# Autodesk Inventor assembly: Center Assembly
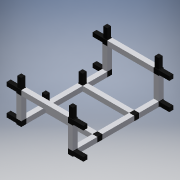
[picture p0: Inventor's stored thumbnail of the model, 180x180]
Saved by Autodesk Inventor 2017 (Build 210142000, 142)
## iProperties
Created: 2019-12-06
Part Number: Center Assembly
Document SubType Name: Assembly
Designer: S346553810
Author: S346553810
## Documents named in this file (9)
- \\ad.ocdsb.ca\studenthome\3\S338674153\FRC 2020\FullRobotRefactor\SubFrame\Center Assembly.iam
- \\ad.ocdsb.ca\studenthome\3\S338674153\FRC 2020\FullRobotRefactor\SubFrame\center cross-member.iam
- \\ad.ocdsb.ca\studenthome\3\S338674153\FRC 2020\FullRobotRefactor\SubFrame\1in sq tub - 4.ipt
- \\ad.ocdsb.ca\studenthome\3\S338674153\FRC 2020\FullRobotRefactor\SubFrame\Kipp K0619.ipt
- \\ad.ocdsb.ca\studenthome\3\S338674153\FRC 2020\FullRobotRefactor\SubFrame\1in sq tub - 6.ipt
- \\ad.ocdsb.ca\studenthome\3\S338674153\FRC 2020\FullRobotRefactor\SubFrame\1in sq tub - 4-5.ipt
- \\ad.ocdsb.ca\studenthome\3\S338674153\FRC 2020\FullRobotRefactor\SubFrame\1in sq tub - 6-5.ipt
- \\ad.ocdsb.ca\studenthome\3\S338674153\FRC 2020\FullRobotRefactor\KIPS\Kipp K0618.ipt
- \\ad.ocdsb.ca\studenthome\3\S338674153\FRC 2020\FullRobotRefactor\KIPS\Kipp K0620.ipt
## Components (14 placed, 8 different names)
1. center cross-member:1 [sub-assembly] — Flush:13, Flush:14, Mate:7
2. 1in sq tub - 4:1 — Flush:12
3. 1in sq tub - 4:2 — Flush:9, Mate:5
4. Kipp K0619:1
5. Kipp K0619:2
6. 1in sq tub - 6:1
7. 1in sq tub - 4-5:1
8. 1in sq tub - 4-5:2
9. 1in sq tub - 6:3
10. 1in sq tub - 6-5:1 — Flush:10, Flush:11, Mate:6, Flush:13
11. Kipp K0618:1
12. Kipp K0618:2 — Flush:14, Mate:7
13. Kipp K0620:1 — Flush:9, Flush:10, Mate:5
14. Kipp K0620:2 — Flush:11, Flush:12, Mate:6
## Relationships (15: Flush 10, Mate 5)
- [Flush]: 1in sq tub - 4-5:2 ↔ Kipp K0618:1
- [Flush]: 1in sq tub - 6:3 ↔ Kipp K0618:1
- [Mate]: 1in sq tub - 6:3 ↔ Kipp K0618:1
- [Flush]: 1in sq tub - 4-5:1 ↔ Kipp K0618:2
- [Flush]: 1in sq tub - 4-5:1 ↔ Kipp K0618:2
- [Mate]: 1in sq tub - 4-5:1 ↔ Kipp K0618:2
- Flush:9: 1in sq tub - 4:2 ↔ Kipp K0620:1
- Flush:10: 1in sq tub - 6-5:1 ↔ Kipp K0620:1
- Mate:5: 1in sq tub - 4:2 ↔ Kipp K0620:1
- Flush:11: 1in sq tub - 6-5:1 ↔ Kipp K0620:2
- Flush:12: 1in sq tub - 4:1 ↔ Kipp K0620:2
- Mate:6: 1in sq tub - 6-5:1 ↔ Kipp K0620:2
- Flush:13: center cross-member:1 ↔ 1in sq tub - 6-5:1
- Flush:14: center cross-member:1 ↔ Kipp K0618:2
- Mate:7: center cross-member:1 ↔ Kipp K0618:2
